# Autodesk Inventor assembly: 4x2
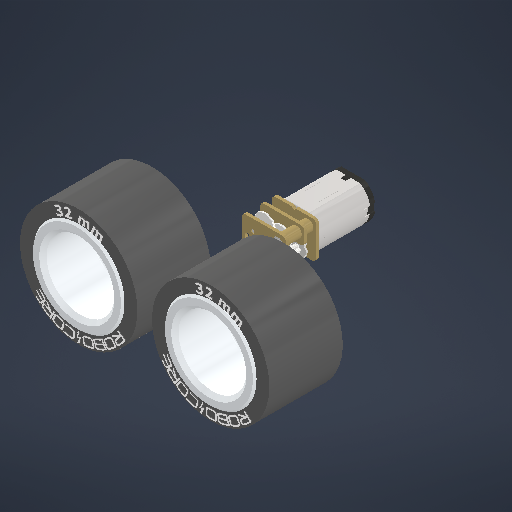
[picture p0: Inventor's stored thumbnail of the model, 512x512]
Saved by Autodesk Inventor 2026.1 (Build 301233020, 233B)
## iProperties
Created: 2026-02-10
Part Number: 4x2
Document SubType Name: Assembly
Designer: celio
Author: celio
## Documents named in this file (3)
- C:\Users\celio\OneDrive\Documentos\Inventor\ZeGuia\Montagem\4x2\Esquema\4x2.iam
- C:\Users\celio\OneDrive\Documentos\Inventor\ZeGuia\Roda\Roda.iam
- C:\Users\celio\OneDrive\Documentos\Inventor\ZeGuia\Motores\N20\N20 DC MOTOR.ipt
## Components (3 placed, 2 different names)
1. Roda:1 [sub-assembly] — Tangente:1, Alinhado:3, Tangente:2, Tangente:4, Tangente:6
2. Roda:2 [sub-assembly] — Tangente:1, Alinhado:2, Tangente:3, Tangente:5
3. N20 DC MOTOR:1 — Coincidente:1, Coincidente:2, Coincidente:3
## Relationships (16: Tangent 6, Angle 3, Mate 3, Flush 2, Symmetry 2)
- Tangente:1 (4 mm): Roda:1 ↔ Roda:2
- Alinhado:2 [Flush]: Roda:2
- Alinhado:3 [Flush]: Roda:1
- Tangente:2: Roda:1
- Tangente:3: Roda:2
- Ângulo:1 [Angle] (0 deg)
- Tangente:4: Roda:1
- Simetria:1 [Symmetry]
- Coincidente:1 [Mate] (-5 mm): N20 DC MOTOR:1
- Ângulo:2 [Angle] (0 deg)
- Tangente:5: Roda:2
- Ângulo:3 [Angle] (0 deg)
- Tangente:6: Roda:1
- Simetria:2 [Symmetry]
- Coincidente:2 [Mate] (12 mm): N20 DC MOTOR:1
- Coincidente:3 [Mate] (-6 mm): N20 DC MOTOR:1
